# Autodesk Inventor assembly: Solenoid
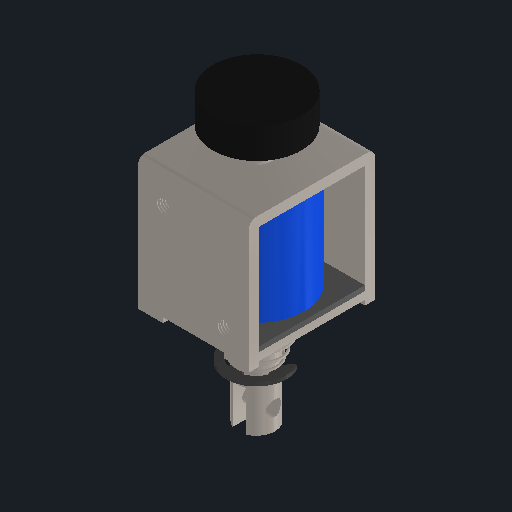
[picture p0: Inventor's stored thumbnail of the model, 512x512]
Saved by Autodesk Inventor 2026.1 (Build 301233020, 233B)
## iProperties
Created: 2025-11-08
Part Number: Solenoid
Document SubType Name: Assembly
Designer: Bahaa
Author: Bahaa
## Documents named in this file (4)
- C:\Users\Bahaa\Nextcloud2\CAD\25-26\Solenoid.iam
- C:\Users\Bahaa\Nextcloud2\CAD\25-26\Solenoid JF-0826B\Solenoid JF-0826B\Solenoid JF-0826B.ipt
- C:\Users\Bahaa\Nextcloud2\CAD\25-26\Solenoid Shield.ipt
- C:\Users\Bahaa\Documents\Inventor\Content Center Files\R2026\en-US\DIN 934\DIN 934 - M3 x 0,5.ipt
## Components (3 placed, 3 different names)
1. Solenoid JF-0826B:1 — Mate:5, Mate:6
2. Solenoid Shield:1 — Mate:1, Mate:2, Mate:3, Mate:6
3. DIN 934 - replaced by DIN EN 24032/28673/28674 M3:2 — Mate:1, Mate:2, Mate:3, Mate:5
## Relationships (5: Mate 5)
- Mate:1: Solenoid Shield:1 ↔ DIN 934 - replaced by DIN EN 24032/28673/28674 M3:2
- Mate:2 (0.025 mm): Solenoid Shield:1 ↔ DIN 934 - replaced by DIN EN 24032/28673/28674 M3:2
- Mate:3 (0.025 mm): Solenoid Shield:1 ↔ DIN 934 - replaced by DIN EN 24032/28673/28674 M3:2
- Mate:5: Solenoid JF-0826B:1 ↔ DIN 934 - replaced by DIN EN 24032/28673/28674 M3:2
- Mate:6: Solenoid JF-0826B:1 ↔ Solenoid Shield:1
